# Autodesk Inventor assembly: Assembly_Guinardia_V0
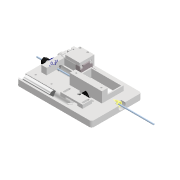
[picture p0: Inventor's stored thumbnail of the model, 180x180]
Saved by Autodesk Inventor 2022 (Build 260153000, 153)
## iProperties
Created: 2022-04-18
Part Number: Assembly_Guinardia_V0
Document SubType Name: Assembly
Designer: Prakash Lab
Author: Prakash Lab
## Documents named in this file (15)
- C:\Users\PrakashLab\Documents\Inventor\Guinardia\INVENTOR\Assembly_Guinardia_V0.iam
- C:\Users\PrakashLab\Documents\Inventor\Guinardia\INVENTOR\00_NEMA8.ipt
- C:\Users\PrakashLab\Documents\Inventor\Guinardia\INVENTOR\10_Wellplate_base.ipt
- C:\Users\PrakashLab\Documents\Inventor\Guinardia\INVENTOR\00_CCTV_lens_M12_25mm_5mp.ipt
- C:\Users\PrakashLab\Documents\Inventor\Guinardia\INVENTOR\00_coverslip_24x50mm.ipt
- C:\Users\PrakashLab\Documents\Inventor\Guinardia\INVENTOR\00_PipetteTip200ul-1.ipt
- C:\Users\PrakashLab\Documents\Inventor\Guinardia\INVENTOR\00_FEP_tube_2.2x0.5mm.ipt
- C:\Users\PrakashLab\Documents\Inventor\Guinardia\INVENTOR\00_Bluraymirror_6.4x6.4x2mm.ipt
- C:\Users\PrakashLab\Documents\Inventor\Guinardia\INVENTOR\00_Laserpointer.ipt
- C:\Users\PrakashLab\Documents\Inventor\Guinardia\INVENTOR\20_Cube_Insert_Lightsheet_FEPTube_Rotating_hollomotor_v0.ipt
- C:\Users\PrakashLab\Documents\Inventor\Guinardia\INVENTOR\00_Bearing_US.ipt
- C:\Users\PrakashLab\Documents\Inventor\Guinardia\INVENTOR\20_Cube_Insert_Lightsheet_FEPTube_Rotating_hollomotor_driver_v0.ipt
- C:\Users\PrakashLab\Documents\Inventor\Guinardia\INVENTOR\00_selfcenter_2mm_nut_v1.ipt
- C:\Users\PrakashLab\Documents\Inventor\Guinardia\INVENTOR\10_LED_cylnderlensmount.ipt
- C:\Users\PrakashLab\Documents\Inventor\Guinardia\INVENTOR\10_Motormount.ipt
## Components (16 placed, 14 different names)
1. 00_NEMA8:1 — Flush:3, Flush:4, Flush:5, Flush:6, Flush:9, Flush:12
2. 10_Wellplate_base:1 — Mate:1, Mate:2, Mate:3, Mate:4, Mate:5, Angle:1, Flush:1, Mate:10, Flush:2, Mate:11, Mate:12, Mate:14, Mate:15, Insert:1, Flush:3, Flush:4, Flush:5, Flush:6, Insert:2, Insert:3, Flush:7, Flush:8, Insert:4, Flush:10, Flush:11
3. 00_CCTV_lens_M12_25mm_5mp:1 — Mate:6, Angle:1, Flush:1
4. 00_coverslip_24x50mm:1 — Mate:1, Mate:2, Mate:3, Mate:7, Mate:13
5. 00_PipetteTip200ul-1:2 — Mate:9, Flush:2
6. 00_FEP_tube_2.2x0.5mm:1 — Mate:4, Mate:5, Mate:8, Mate:9, Mate:7
7. 00_PipetteTip200ul-1:3 — Mate:8, Mate:6, Mate:10
8. 00_coverslip_24x50mm:2 — Mate:11, Mate:12, Mate:13
9. 00_Bluraymirror_6.4x6.4x2mm:1 — Mate:14, Mate:15
10. 00_Laserpointer:1 — Insert:1
11. 20_Cube_Insert_Lightsheet_FEPTube_Rotating_hollomotor_v0:1 — Insert:2
12. 00_Bearing_US:1 — Insert:3
13. 20_Cube_Insert_Lightsheet_FEPTube_Rotating_hollomotor_driver_v0:1 — Flush:7, Flush:8, Flush:9
14. 00_selfcenter_2mm_nut_v1:1 — Insert:4
15. 10_LED_cylnderlensmount:1 — Flush:10, Flush:11
16. 10_Motormount:1 — Flush:12
## Relationships (32: Mate 15, Flush 12, Insert 4, Angle 1)
- Mate:1: 10_Wellplate_base:1 ↔ 00_coverslip_24x50mm:1
- Mate:2: 10_Wellplate_base:1 ↔ 00_coverslip_24x50mm:1
- Mate:3: 10_Wellplate_base:1 ↔ 00_coverslip_24x50mm:1
- Mate:4 (-6 mm): 10_Wellplate_base:1 ↔ 00_FEP_tube_2.2x0.5mm:1
- Mate:5: 10_Wellplate_base:1 ↔ 00_FEP_tube_2.2x0.5mm:1
- Mate:8: 00_FEP_tube_2.2x0.5mm:1 ↔ 00_PipetteTip200ul-1:3
- Mate:9: 00_PipetteTip200ul-1:2 ↔ 00_FEP_tube_2.2x0.5mm:1
- Mate:6: 00_CCTV_lens_M12_25mm_5mp:1 ↔ 00_PipetteTip200ul-1:3
- Angle:1 (0 deg): 10_Wellplate_base:1 ↔ 00_CCTV_lens_M12_25mm_5mp:1
- Flush:1: 10_Wellplate_base:1 ↔ 00_CCTV_lens_M12_25mm_5mp:1
- Mate:7 (3 mm): 00_coverslip_24x50mm:1 ↔ 00_FEP_tube_2.2x0.5mm:1
- Mate:10 (4 mm): 10_Wellplate_base:1 ↔ 00_PipetteTip200ul-1:3
- Flush:2 (5 mm): 10_Wellplate_base:1 ↔ 00_PipetteTip200ul-1:2
- Mate:11: 10_Wellplate_base:1 ↔ 00_coverslip_24x50mm:2
- Mate:12: 10_Wellplate_base:1 ↔ 00_coverslip_24x50mm:2
- Mate:13: 00_coverslip_24x50mm:1 ↔ 00_coverslip_24x50mm:2
- Mate:14: 10_Wellplate_base:1 ↔ 00_Bluraymirror_6.4x6.4x2mm:1
- Mate:15: 10_Wellplate_base:1 ↔ 00_Bluraymirror_6.4x6.4x2mm:1
- Insert:1: 10_Wellplate_base:1 ↔ 00_Laserpointer:1
- Flush:3 (1 mm): 00_NEMA8:1 ↔ 10_Wellplate_base:1
- Flush:4 (5 mm): 00_NEMA8:1 ↔ 10_Wellplate_base:1
- Flush:5 (16 mm): 00_NEMA8:1 ↔ 10_Wellplate_base:1
- Flush:6: 00_NEMA8:1 ↔ 10_Wellplate_base:1
- Insert:2: 10_Wellplate_base:1 ↔ 20_Cube_Insert_Lightsheet_FEPTube_Rotating_hollomotor_v0:1
- Insert:3: 10_Wellplate_base:1 ↔ 00_Bearing_US:1
- Flush:7: 10_Wellplate_base:1 ↔ 20_Cube_Insert_Lightsheet_FEPTube_Rotating_hollomotor_driver_v0:1
- Flush:8: 10_Wellplate_base:1 ↔ 20_Cube_Insert_Lightsheet_FEPTube_Rotating_hollomotor_driver_v0:1
- Flush:9: 00_NEMA8:1 ↔ 20_Cube_Insert_Lightsheet_FEPTube_Rotating_hollomotor_driver_v0:1
- Insert:4: 10_Wellplate_base:1 ↔ 00_selfcenter_2mm_nut_v1:1
- Flush:10: 10_Wellplate_base:1 ↔ 10_LED_cylnderlensmount:1
- Flush:11: 10_Wellplate_base:1 ↔ 10_LED_cylnderlensmount:1
- Flush:12: 00_NEMA8:1 ↔ 10_Motormount:1
